# Autodesk Inventor assembly: Knee
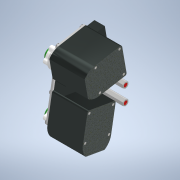
[picture p0: Inventor's stored thumbnail of the model, 180x180]
Saved by Autodesk Inventor 2020 (Build 240168000, 168)
## iProperties
Created: 2021-09-06
Part Number: Knee
Document SubType Name: Assembly
Designer: Masato
Mass: 264.861 g
Surface Area: 473.637 cm^2
Volume: 130.531 cm^3
Density: 2.0291 g/cm^3
Author: Masato
## Documents named in this file (15)
- C:\Users\Masato\Documents\Inventor\CIT Brains_Inventor\OpenPlatform_ver3_0 - Ver4_1branch\LowerBody\Knee\Knee.iam
- C:\Users\Masato\Documents\Inventor\CIT Brains_Inventor\OpenPlatform_ver3_0 - Ver4_1branch\LowerBody\Knee\Knee_side_frame.ipt
- C:\Users\Masato\Documents\Inventor\CIT Brains_Inventor\OpenPlatform_ver3_0\Ready_Made\B3M11xx.ipt
- C:\Users\Masato\Documents\Inventor\CIT Brains_Inventor\OpenPlatform_ver3_0 - Ver4_1branch\LowerBody\Knee\Knee_clamp.ipt
- C:\Users\Masato\Documents\Inventor\CIT Brains_Inventor\OpenPlatform_ver3_0\Ready_Made\FreeHorn.ipt
- C:\Users\Masato\Documents\Inventor\CIT Brains_Inventor\OpenPlatform_ver3_0\Ready_Made\WSSS-12-10-8.ipt
- C:\Users\Masato\Documents\Inventor\CIT Brains_Inventor\OpenPlatform_ver3_0\Ready_Made\80F-0603.ipt
- C:\Users\Masato\Documents\Inventor\CIT Brains_Inventor\OpenPlatform_ver3_0 - Ver4_1branch\Ready_Made\Screw\M2_6-15.ipt
- C:\Users\Masato\Documents\Inventor\CIT Brains_Inventor\OpenPlatform_ver3_0 - Ver4_1branch\Ready_Made\Screw\M2_6-20.ipt
- C:\Users\Masato\Documents\Inventor\CIT Brains_Inventor\OpenPlatform_ver3_0\Ready_Made\CC-0612-15B.ipt
- C:\Users\Masato\Documents\Inventor\CIT Brains_Inventor\OpenPlatform_ver3_0\Ready_Made\CC-0612-50B.ipt
- C:\Users\Masato\Documents\Inventor\CIT Brains_Inventor\OpenPlatform_ver3_0 - Ver4_1branch\Ready_Made\Screw\FreeHorn_Screw.ipt
- C:\Users\Masato\Documents\Inventor\CIT Brains_Inventor\OpenPlatform_ver3_0 - Ver4_1branch\Ready_Made\SLSBF6-39_5-M4-N4.ipt
- C:\Users\Masato\Documents\Inventor\CIT Brains_Inventor\OpenPlatform_ver3_0 - Ver4_1branch\Ready_Made\DBTS4-11-6.ipt
- C:\Users\Masato\Documents\Inventor\CIT Brains_Inventor\OpenPlatform_ver3_0 - Ver4_1branch\Ready_Made\UUW-0412-10BH.ipt
## Components (54 placed, 14 different names)
1. Knee_side_frame:1 — 挿入:1, 挿入:2, 挿入:3, 挿入:4, 挿入:5, 挿入:6, 挿入:7, 挿入:8, フラッシュ:4, フラッシュ:6, 挿入:93, 挿入:94, 挿入:95, 挿入:96, 挿入:97, 挿入:98, 挿入:99, 挿入:100, 挿入:114, 挿入:115, 挿入:121, 挿入:122
2. Knee_side_frame:2 — 挿入:9, 挿入:10, 挿入:11, 挿入:12, 挿入:13, 挿入:14, 挿入:15, 挿入:16, 挿入:85, 挿入:86, 挿入:87, 挿入:88, 挿入:89, 挿入:90, 挿入:91, 挿入:92, 挿入:116, 挿入:117, 挿入:119, 挿入:120
3. B3M11xx:1 — 挿入:1, 挿入:2, 挿入:5, 挿入:6, 挿入:9, 挿入:10, 挿入:15, 挿入:16, 挿入:31, 挿入:33, 挿入:112, 挿入:132
4. B3M11xx:2 — 挿入:3, 挿入:4, 挿入:7, 挿入:8, 挿入:11, 挿入:12, 挿入:13, 挿入:14, 挿入:32, 挿入:34, 挿入:113, 挿入:131
5. Knee_clamp:1 — 挿入:32, 挿入:61, 挿入:131, メイト:2
6. Knee_clamp:2 — 挿入:31, 挿入:62, 挿入:132, メイト:1
7. Knee_clamp:3 — 挿入:36, 挿入:63, メイト:2, 挿入:133
8. Knee_clamp:4 — 挿入:35, 挿入:64, メイト:1, 挿入:134
9. FreeHorn:1 — 挿入:33, 挿入:35, 挿入:134
10. FreeHorn:2 — 挿入:34, 挿入:36, 挿入:133
11. WSSS-12-10-8:1 — 挿入:64
12. WSSS-12-10-8:2 — 挿入:63
13. WSSS-12-10-8:3 — 挿入:62
14. WSSS-12-10-8:4 — 挿入:61
15. 80F-0603:1 — 挿入:110
16. 80F-0603:2 — 挿入:109
17. 80F-0603:3 — 挿入:118
18. 80F-0603:4 — 挿入:111
19. M2_6-15:1 — 挿入:85
20. M2_6-15:2 — 挿入:86
21. M2_6-15:3 — 挿入:87
22. M2_6-15:4 — 挿入:88
23. M2_6-15:5 — 挿入:89
24. M2_6-15:6 — 挿入:90
25. M2_6-15:7 — 挿入:91
26. M2_6-15:8 — 挿入:92
27. M2_6-20:1 — 挿入:93
28. M2_6-20:2 — 挿入:94
29. M2_6-20:3 — 挿入:95
30. M2_6-20:4 — 挿入:96
31. M2_6-20:5 — 挿入:97
32. M2_6-20:6 — 挿入:98
33. M2_6-20:7 — 挿入:99
34. M2_6-20:8 — 挿入:100
35. CC-0612-15B:1 — 挿入:101, 挿入:126
36. CC-0612-15B:2 — 挿入:102, 挿入:125
37. CC-0612-15B:3 — 挿入:103, 挿入:123
38. CC-0612-15B:4 — 挿入:104, 挿入:124
39. CC-0612-50B:1 — 挿入:101, 挿入:118
40. CC-0612-50B:2 — 挿入:102, 挿入:111
41. CC-0612-50B:3 — 挿入:103, 挿入:109
42. CC-0612-50B:4 — 挿入:104, 挿入:110
43. FreeHorn_Screw:1 — 挿入:112
44. FreeHorn_Screw:2 — 挿入:113
45. SLSBF6-39_5-M4-N4:1 — 挿入:114, 挿入:116, 角度:2
46. SLSBF6-39_5-M4-N4:2 — 挿入:115, 挿入:117, 角度:2
47. DBTS4-11-6:1 — 挿入:130
48. DBTS4-11-6:2 — 挿入:129
49. DBTS4-11-6:3 — 挿入:128
50. DBTS4-11-6:4 — 挿入:127
51. UUW-0412-10BH:1 — 挿入:119, 挿入:125, 挿入:127
52. UUW-0412-10BH:2 — 挿入:120, 挿入:126, 挿入:128
53. UUW-0412-10BH:3 — 挿入:121, 挿入:123, 挿入:129
54. UUW-0412-10BH:4 — 挿入:122, 挿入:124, 挿入:130
## Relationships (77: Insert 72, Flush 2, Mate 2, Angle 1)
- 挿入:1 [Insert]: Knee_side_frame:1 ↔ B3M11xx:1
- 挿入:2 [Insert]: Knee_side_frame:1 ↔ B3M11xx:1
- 挿入:3 [Insert]: Knee_side_frame:1 ↔ B3M11xx:2
- 挿入:4 [Insert]: Knee_side_frame:1 ↔ B3M11xx:2
- 挿入:5 [Insert]: Knee_side_frame:1 ↔ B3M11xx:1
- 挿入:6 [Insert]: Knee_side_frame:1 ↔ B3M11xx:1
- 挿入:7 [Insert]: Knee_side_frame:1 ↔ B3M11xx:2
- 挿入:8 [Insert]: Knee_side_frame:1 ↔ B3M11xx:2
- 挿入:9 [Insert]: Knee_side_frame:2 ↔ B3M11xx:1
- 挿入:10 [Insert]: Knee_side_frame:2 ↔ B3M11xx:1
- 挿入:11 [Insert]: Knee_side_frame:2 ↔ B3M11xx:2
- 挿入:12 [Insert]: Knee_side_frame:2 ↔ B3M11xx:2
- 挿入:13 [Insert]: Knee_side_frame:2 ↔ B3M11xx:2
- 挿入:14 [Insert]: Knee_side_frame:2 ↔ B3M11xx:2
- 挿入:15 [Insert]: Knee_side_frame:2 ↔ B3M11xx:1
- 挿入:16 [Insert]: Knee_side_frame:2 ↔ B3M11xx:1
- 挿入:31 [Insert]: B3M11xx:1 ↔ Knee_clamp:2
- 挿入:32 [Insert]: B3M11xx:2 ↔ Knee_clamp:1
- 挿入:33 [Insert]: B3M11xx:1 ↔ FreeHorn:1
- 挿入:34 [Insert]: B3M11xx:2 ↔ FreeHorn:2
- 挿入:35 [Insert]: Knee_clamp:4 ↔ FreeHorn:1
- 挿入:36 [Insert]: Knee_clamp:3 ↔ FreeHorn:2
- フラッシュ:4 [Flush] (-19.75 mm): Knee_side_frame:1
- 挿入:61 [Insert]: Knee_clamp:1 ↔ WSSS-12-10-8:4
- 挿入:62 [Insert]: Knee_clamp:2 ↔ WSSS-12-10-8:3
- 挿入:63 [Insert]: Knee_clamp:3 ↔ WSSS-12-10-8:2
- 挿入:64 [Insert]: Knee_clamp:4 ↔ WSSS-12-10-8:1
- フラッシュ:6 [Flush]: Knee_side_frame:1
- 挿入:85 [Insert]: Knee_side_frame:2 ↔ M2_6-15:1
- 挿入:86 [Insert]: Knee_side_frame:2 ↔ M2_6-15:2
- 挿入:87 [Insert]: Knee_side_frame:2 ↔ M2_6-15:3
- 挿入:88 [Insert]: Knee_side_frame:2 ↔ M2_6-15:4
- 挿入:89 [Insert]: Knee_side_frame:2 ↔ M2_6-15:5
- 挿入:90 [Insert]: Knee_side_frame:2 ↔ M2_6-15:6
- 挿入:91 [Insert]: Knee_side_frame:2 ↔ M2_6-15:7
- 挿入:92 [Insert]: Knee_side_frame:2 ↔ M2_6-15:8
- 挿入:93 [Insert]: Knee_side_frame:1 ↔ M2_6-20:1
- 挿入:94 [Insert]: Knee_side_frame:1 ↔ M2_6-20:2
- 挿入:95 [Insert]: Knee_side_frame:1 ↔ M2_6-20:3
- 挿入:96 [Insert]: Knee_side_frame:1 ↔ M2_6-20:4
- 挿入:97 [Insert]: Knee_side_frame:1 ↔ M2_6-20:5
- 挿入:98 [Insert]: Knee_side_frame:1 ↔ M2_6-20:6
- 挿入:99 [Insert]: Knee_side_frame:1 ↔ M2_6-20:7
- 挿入:100 [Insert]: Knee_side_frame:1 ↔ M2_6-20:8
- 挿入:101 [Insert]: CC-0612-15B:1 ↔ CC-0612-50B:1
- 挿入:102 [Insert]: CC-0612-15B:2 ↔ CC-0612-50B:2
- 挿入:103 [Insert]: CC-0612-15B:3 ↔ CC-0612-50B:3
- 挿入:104 [Insert]: CC-0612-15B:4 ↔ CC-0612-50B:4
- 挿入:109 [Insert]: 80F-0603:2 ↔ CC-0612-50B:3
- 挿入:110 [Insert]: 80F-0603:1 ↔ CC-0612-50B:4
- 挿入:111 [Insert]: 80F-0603:4 ↔ CC-0612-50B:2
- 挿入:112 [Insert]: B3M11xx:1 ↔ FreeHorn_Screw:1
- 挿入:113 [Insert]: B3M11xx:2 ↔ FreeHorn_Screw:2
- 挿入:114 [Insert]: Knee_side_frame:1 ↔ SLSBF6-39_5-M4-N4:1
- 挿入:115 [Insert]: Knee_side_frame:1 ↔ SLSBF6-39_5-M4-N4:2
- 挿入:116 [Insert]: Knee_side_frame:2 ↔ SLSBF6-39_5-M4-N4:1
- 挿入:117 [Insert]: Knee_side_frame:2 ↔ SLSBF6-39_5-M4-N4:2
- 角度:2 [Angle] (0 deg): SLSBF6-39_5-M4-N4:1 ↔ SLSBF6-39_5-M4-N4:2
- 挿入:118 [Insert]: 80F-0603:3 ↔ CC-0612-50B:1
- 挿入:119 [Insert]: Knee_side_frame:2 ↔ UUW-0412-10BH:1
- 挿入:120 [Insert]: Knee_side_frame:2 ↔ UUW-0412-10BH:2
- 挿入:121 [Insert]: Knee_side_frame:1 ↔ UUW-0412-10BH:3
- 挿入:122 [Insert]: Knee_side_frame:1 ↔ UUW-0412-10BH:4
- 挿入:123 [Insert]: CC-0612-15B:3 ↔ UUW-0412-10BH:3
- 挿入:124 [Insert]: CC-0612-15B:4 ↔ UUW-0412-10BH:4
- 挿入:125 [Insert]: CC-0612-15B:2 ↔ UUW-0412-10BH:1
- 挿入:126 [Insert]: CC-0612-15B:1 ↔ UUW-0412-10BH:2
- 挿入:127 [Insert]: DBTS4-11-6:4 ↔ UUW-0412-10BH:1
- 挿入:128 [Insert]: DBTS4-11-6:3 ↔ UUW-0412-10BH:2
- 挿入:129 [Insert]: DBTS4-11-6:2 ↔ UUW-0412-10BH:3
- 挿入:130 [Insert]: DBTS4-11-6:1 ↔ UUW-0412-10BH:4
- 挿入:131 [Insert]: B3M11xx:2 ↔ Knee_clamp:1
- 挿入:132 [Insert]: B3M11xx:1 ↔ Knee_clamp:2
- メイト:1 [Mate]: Knee_clamp:2 ↔ Knee_clamp:4
- メイト:2 [Mate]: Knee_clamp:1 ↔ Knee_clamp:3
- 挿入:133 [Insert]: Knee_clamp:3 ↔ FreeHorn:2
- 挿入:134 [Insert]: Knee_clamp:4 ↔ FreeHorn:1
